# Autodesk Inventor assembly: Arduino and Pi assembly
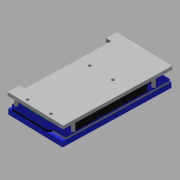
[picture p0: Inventor's stored thumbnail of the model, 180x180]
Saved by Autodesk Inventor 2017 (Build 210142000, 142)
## iProperties
Created: 2017-01-13
Part Number: Arduino and Pi assembly
Document SubType Name: Assembly
Designer: qupec
Author: qupec
## Documents named in this file (5)
- C:\Users\qupec\Desktop\UMD Near Space\RockSat\Arduino and Pi assembly.iam
- C:\Users\qupec\Desktop\UMD Near Space\RockSat\Arduino Mount.ipt
- C:\Users\qupec\Desktop\UMD Near Space\RockSat\Arduino Mega.ipt
- C:\Users\qupec\Desktop\UMD Near Space\RockSat\Pi Holder.ipt
- C:\Users\qupec\Desktop\UMD Near Space\RockSat\Pi Cam\RapberryPiZero.ipt
## Components (4 placed, 4 different names)
1. Arduino Mount:1 — Mate:3, Flush:1, Mate:7, Mate:8
2. Arduino Mega:1 — Mate:3, Mate:5
3. Pi Holder:1 — Flush:1, Mate:5, Mate:6, Mate:7, Mate:8, Flush:2, Mate:9
4. RapberryPiZero:1 — Mate:6, Flush:2, Mate:9
## Relationships (8: Mate 6, Flush 2)
- Mate:3: Arduino Mount:1 ↔ Arduino Mega:1
- Flush:1: Arduino Mount:1 ↔ Pi Holder:1
- Mate:5: Arduino Mega:1 ↔ Pi Holder:1
- Mate:6: Pi Holder:1 ↔ RapberryPiZero:1
- Mate:7: Arduino Mount:1 ↔ Pi Holder:1
- Mate:8: Arduino Mount:1 ↔ Pi Holder:1
- Flush:2: Pi Holder:1 ↔ RapberryPiZero:1
- Mate:9: Pi Holder:1 ↔ RapberryPiZero:1
